# Autodesk Inventor assembly: linear_cutting_endeffector_idea
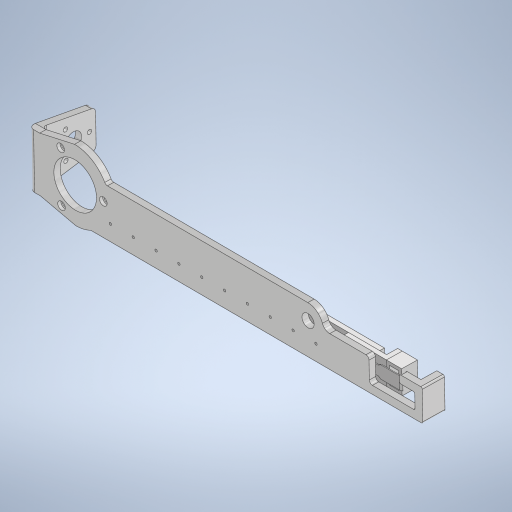
[picture p0: Inventor's stored thumbnail of the model, 512x512]
Saved by Autodesk Inventor 2024 (Build 280153000, 153)
## iProperties
Created: 2025-06-10
Part Number: linear_cutting_endeffector_idea
Document SubType Name: Assembly
Designer: 1412z
Author: 1412z
## Documents named in this file (12)
- C:\Users\1412z\OneDrive\デスクトップ\rdclab\harvesting_robot\harvesting_endeffector\linear_cutting_endeffector\linear_cutting_endeffector_idea.iam
- C:\Users\1412z\OneDrive\デスクトップ\rdclab\harvesting_robot\harvesting_endeffector\linear_cutting_endeffector\misumi\LRGEAM0.8KA-80-K2-B50_Autodesk_Inventor_2024_20250607\LRGEAM0_8KA-80-K2-B50.ipt
- C:\Users\1412z\OneDrive\デスクトップ\rdclab\harvesting_robot\harvesting_endeffector\linear_cutting_endeffector\misumi\pipe\Φ3.6-Φ2.2-4.ipt
- C:\Users\1412z\OneDrive\デスクトップ\rdclab\harvesting_robot\harvesting_endeffector\linear_cutting_endeffector\misumi\washer\washer_M2.ipt
- C:\Users\1412z\OneDrive\デスクトップ\rdclab\harvesting_robot\harvesting_endeffector\linear_cutting_endeffector\misumi\screw\M2×6\M2×6.ipt
- C:\Users\1412z\OneDrive\デスクトップ\rdclab\harvesting_robot\harvesting_endeffector\claws_endeffector\cutter_part\pen_type_cutter.ipt
- C:\Users\1412z\OneDrive\デスクトップ\rdclab\harvesting_robot\harvesting_endeffector\linear_slider\AIS2024\SSEB6L-145-B3.iam
- C:\Users\1412z\OneDrive\デスクトップ\rdclab\harvesting_robot\harvesting_endeffector\linear_cutting_endeffector\cutter\cutter_holder.ipt
- C:\Users\1412z\OneDrive\デスクトップ\rdclab\harvesting_robot\harvesting_endeffector\linear_cutting_endeffector\cutter\sponge_holder.ipt
- C:\Users\1412z\OneDrive\デスクトップ\rdclab\harvesting_robot\harvesting_endeffector\linear_cutting_endeffector\cutter\slider_to_cutter_part.ipt
- C:\Users\1412z\OneDrive\デスクトップ\rdclab\harvesting_robot\harvesting_endeffector\linear_cutting_endeffector\cutter\sponge.ipt
- C:\Users\1412z\OneDrive\デスクトップ\rdclab\harvesting_robot\harvesting_endeffector\linear_cutting_endeffector\motor_holder\motor_holder-3.ipt
## Components (14 placed, 11 different names)
1. pen_type_cutter:1 — メイト:1, メイト:2, メイト:3
2. SSEB6L-145-B3:2 [sub-assembly] — 挿入:9, 挿入:10, 挿入:11, 挿入:12, 挿入:15, 挿入:18
3. cutter_holder:1 — メイト:1, メイト:2, 挿入:3, 挿入:4, メイト:3
4. sponge_holder:1 — 挿入:3, 挿入:4, 挿入:7, 挿入:8, 挿入:13, 挿入:14
5. slider_to_cutter_part:1 — 挿入:7, 挿入:8, 挿入:9, 挿入:10, 挿入:15, 挿入:18, 挿入:19, 挿入:20
6. sponge:1 — 挿入:13, 挿入:14
7. motor_holder-3:1 — 挿入:11, 挿入:12
8. LRGEAM0_8KA-80-K2-B50:3 — 挿入:19, 挿入:20
9. Φ3.6-Φ2.2-4:5
10. washer_M2:5
11. M2×6:5
12. Φ3.6-Φ2.2-4:6
13. washer_M2:6
14. M2×6:6
## Relationships (23: Insert 16, RevoluteJoint 4, Mate 3)
- メイト:1 [Mate]: pen_type_cutter:1 ↔ cutter_holder:1
- メイト:2 [Mate]: pen_type_cutter:1 ↔ cutter_holder:1
- 挿入:3 [Insert]: cutter_holder:1 ↔ sponge_holder:1
- 挿入:4 [Insert]: cutter_holder:1 ↔ sponge_holder:1
- メイト:3 [Mate] (0.5 mm): pen_type_cutter:1 ↔ cutter_holder:1
- 挿入:7 [Insert]: sponge_holder:1 ↔ slider_to_cutter_part:1
- 挿入:8 [Insert]: sponge_holder:1 ↔ slider_to_cutter_part:1
- 挿入:9 [Insert]: SSEB6L-145-B3:2 ↔ slider_to_cutter_part:1
- 挿入:10 [Insert]: SSEB6L-145-B3:2 ↔ slider_to_cutter_part:1
- 挿入:11 [Insert]: SSEB6L-145-B3:2 ↔ motor_holder-3:1
- 挿入:12 [Insert]: SSEB6L-145-B3:2 ↔ motor_holder-3:1
- 挿入:13 [Insert]: sponge_holder:1 ↔ sponge:1
- 挿入:14 [Insert]: sponge_holder:1 ↔ sponge:1
- 挿入:15 [Insert]: SSEB6L-145-B3:2 ↔ slider_to_cutter_part:1
- [RevoluteJoint]: Φ3.6-Φ2.2-4:5 ↔ washer_M2:5
- [RevoluteJoint]: washer_M2:5 ↔ M2×6:5
- [RevoluteJoint]: Φ3.6-Φ2.2-4:6 ↔ washer_M2:6
- [RevoluteJoint]: washer_M2:6 ↔ M2×6:6
- [Insert]: LRGEAM0_8KA-80-K2-B50:3 ↔ Φ3.6-Φ2.2-4:6
- [Insert]: LRGEAM0_8KA-80-K2-B50:3 ↔ Φ3.6-Φ2.2-4:5
- 挿入:18 [Insert]: SSEB6L-145-B3:2 ↔ slider_to_cutter_part:1
- 挿入:19 [Insert]: slider_to_cutter_part:1 ↔ LRGEAM0_8KA-80-K2-B50:3
- 挿入:20 [Insert]: slider_to_cutter_part:1 ↔ LRGEAM0_8KA-80-K2-B50:3
## Named parameters: d150_d124_d122 = 0 mm, d151_d125_d123 = 2.593353 deg, d152_d126_d118 = 0 mm, d153_d127_d119 = 55.514814 deg, d154_d128_d122 = 0 mm, d155_d129_d123 = 2.594597 deg, d156_d130_d118 = 0 mm, d157_d131_d119 = 65.052829 deg, d158_d132 = 0 mm, d159_d133 = 0 mm
